# Autodesk Inventor assembly: ZLLG80ASM250-L V3.0 Single shaft
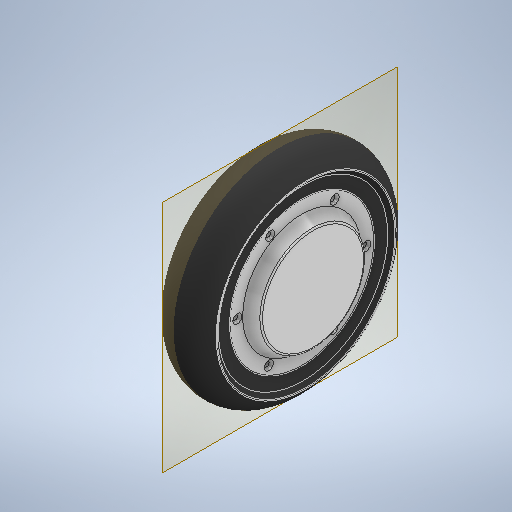
[picture p0: Inventor's stored thumbnail of the model, 512x512]
Saved by Autodesk Inventor 2026.2 (Build 302298010, 298A)
## iProperties
Company: none
Created: 2022-02-19
Part Number: ZLLG80ASM250-L V3.0 Single shaft
Description: CATIA V5 STEP Exchange
Document SubType Name: Assembly
Designer: chanh
Authority: none
Sending System: CATIA V5 STEP AP203
Preprocessor: CATIA Version 5 Release 20 GA (IN-10)
Title: C:\Users\Administrator\Desktop\常规电机图纸\8寸\ZLLG80ASM250 V3.0单出轴\ZLLG80ASM250-L V3.0.stp
Author: none
## Documents named in this file (7)
- C:\Users\chanh\내 드라이브\교과공부\2026년 1학기 (4학년 1학기)\01창의제품설계\CLOSE_hardware\00부품\ZLLG80ASM250-L V3.0 (모터)\ZLLG80ASM250-L V3.0 Single shaft.iam
- C:\Users\chanh\내 드라이브\교과공부\2026년 1학기 (4학년 1학기)\01창의제품설계\CLOSE_hardware\00부품\ZLLG80ASM250-L V3.0 (모터)\shaft.ipt
- C:\Users\chanh\내 드라이브\교과공부\2026년 1학기 (4학년 1학기)\01창의제품설계\CLOSE_hardware\00부품\ZLLG80ASM250-L V3.0 (모터)\outer cover.ipt
- C:\Users\chanh\내 드라이브\교과공부\2026년 1학기 (4학년 1학기)\01창의제품설계\CLOSE_hardware\00부품\ZLLG80ASM250-L V3.0 (모터)\inner ring.ipt
- C:\Users\chanh\내 드라이브\교과공부\2026년 1학기 (4학년 1학기)\01창의제품설계\CLOSE_hardware\00부품\ZLLG80ASM250-L V3.0 (모터)\tire.ipt
- C:\Users\chanh\내 드라이브\교과공부\2026년 1학기 (4학년 1학기)\01창의제품설계\CLOSE_hardware\00부품\ZLLG80ASM250-L V3.0 (모터)\inner cover.ipt
- C:\Users\chanh\내 드라이브\교과공부\2026년 1학기 (4학년 1학기)\01창의제품설계\CLOSE_hardware\00부품\ZLLG80ASM250-L V3.0 (모터)\Washer.ipt
## Components (6 placed, 6 different names)
1. shaft
2. outer cover
3. inner ring
4. tire — Angle:1, Mate:1
5. inner cover
6. Washer
## Relationships (2: Angle 1, Mate 1)
- Angle:1 (0 deg): tire
- Mate:1: tire
